# Autodesk Inventor assembly: Baugruppe1
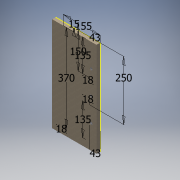
[picture p0: Inventor's stored thumbnail of the model, 180x180]
Saved by Autodesk Inventor 2017.2 (Build 212233000, 233)
## iProperties
Part Number: Baugruppe1
Material: Generisch
Document SubType Name: Assembly
Designer: Daniel
Author: Daniel
## Documents named in this file (4)
- C:\Users\Daniel\Desktop\Autocad\inventor\Baugruppe1.iam
- C:\Users\Daniel\Desktop\Autocad\inventor\frontHolz.ipt
- C:\Users\Daniel\Desktop\Autocad\inventor\schrauben\211309-4_5x25_17.ipt
- C:\Users\Daniel\Desktop\Autocad\inventor\schrauben\din_en_iso2009_m6x25_4_8.ipt
## Components (11 placed, 3 different names)
1. frontHolz:1 — Einfügen:1, Einfügen:2, Einfügen:3, Einfügen:4, Einfügen:5, Einfügen:6, Einfügen:7, Einfügen:8, Einfügen:9, Einfügen:10
2. 211309-4_5x25_17:1 — Einfügen:1
3. 211309-4_5x25_17:2 — Einfügen:4
4. 211309-4_5x25_17:3 — Einfügen:5
5. 211309-4_5x25_17:4 — Einfügen:3
6. 211309-4_5x25_17:5 — Einfügen:2
7. 211309-4_5x25_17:6 — Einfügen:6
8. 211309-4_5x25_17:7 — Einfügen:7
9. din_en_iso2009_m6x25_4_8:1 — Einfügen:9
10. din_en_iso2009_m6x25_4_8:2 — Einfügen:10
11. din_en_iso2009_m6x25_4_8:3 — Einfügen:8
## Relationships (10: Insert 10)
- Einfügen:1 [Insert]: frontHolz:1 ↔ 211309-4_5x25_17:1
- Einfügen:2 [Insert]: frontHolz:1 ↔ 211309-4_5x25_17:5
- Einfügen:3 [Insert]: frontHolz:1 ↔ 211309-4_5x25_17:4
- Einfügen:4 [Insert]: frontHolz:1 ↔ 211309-4_5x25_17:2
- Einfügen:5 [Insert]: frontHolz:1 ↔ 211309-4_5x25_17:3
- Einfügen:6 [Insert]: frontHolz:1 ↔ 211309-4_5x25_17:6
- Einfügen:7 [Insert]: frontHolz:1 ↔ 211309-4_5x25_17:7
- Einfügen:8 [Insert]: frontHolz:1 ↔ din_en_iso2009_m6x25_4_8:3
- Einfügen:9 [Insert]: frontHolz:1 ↔ din_en_iso2009_m6x25_4_8:1
- Einfügen:10 [Insert]: frontHolz:1 ↔ din_en_iso2009_m6x25_4_8:2
